# Autodesk Inventor assembly: BRACER ASSEMBLIES
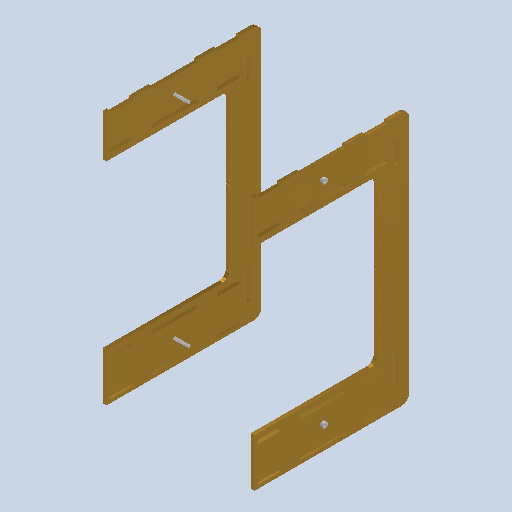
[picture p0: Inventor's stored thumbnail of the model, 512x512]
Saved by Autodesk Inventor 2022.2 (Build 262287010, 287A)
## iProperties
Created: 2021-06-17
Part Number: BRACER ASSEMBLIES
Document SubType Name: Assembly
Designer: benka
Author: benka
## Documents named in this file (3)
- C:\Users\benka\University College London\AHRC - PBD Exhibitions - UCL_Code(Development) - UCL_Code(All)\0.Board Manufacturing&Box building\1.In-home manufacturing\PBD case\1x1 slim\Model\BRACER ASSEMBLIES.iam
- C:\Users\benka\University College London\AHRC - PBD Exhibitions - UCL_Code(Development) - UCL_Code(All)\0.Board Manufacturing&Box building\1.In-home manufacturing\PBD case\1x1 slim\Model\ipt\side bracer.ipt
- C:\Users\benka\University College London\AHRC - PBD Exhibitions - UCL_Code(Development) - UCL_Code(All)\0.Board Manufacturing&Box building\1.In-home manufacturing\PBD case\1x1 slim\Model\ipt\M4 Hex Screw v2 - 25.ipt
## Components (6 placed, 2 different names)
1. side bracer:1 — Mate:6, Mate:7, Mate:8, Mate:9
2. side bracer:2 — Mate:10, Mate:11
3. M4 Hex Screw v2 - 25:1 — Mate:6, Mate:9
4. M4 Hex Screw v2 - 25:2 — Mate:7, Mate:8
5. M4 Hex Screw v2 - 25:3 — Mate:11
6. M4 Hex Screw v2 - 25:4 — Mate:10
## Relationships (6: Mate 6)
- Mate:6: side bracer:1 ↔ M4 Hex Screw v2 - 25:1
- Mate:7: side bracer:1 ↔ M4 Hex Screw v2 - 25:2
- Mate:8: side bracer:1 ↔ M4 Hex Screw v2 - 25:2
- Mate:9: side bracer:1 ↔ M4 Hex Screw v2 - 25:1
- Mate:10: side bracer:2 ↔ M4 Hex Screw v2 - 25:4
- Mate:11: side bracer:2 ↔ M4 Hex Screw v2 - 25:3
